# Autodesk Inventor assembly: rear_sled
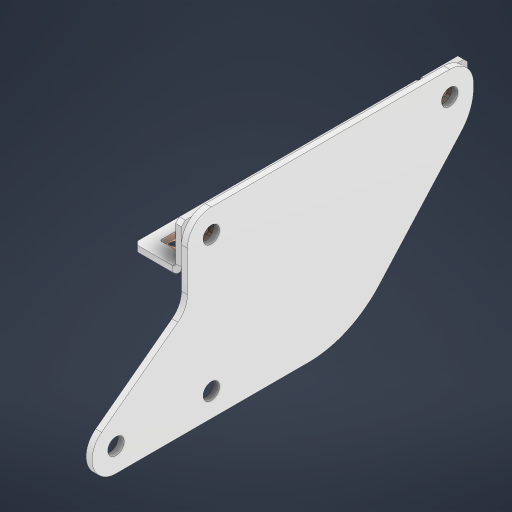
[picture p0: Inventor's stored thumbnail of the model, 512x512]
Saved by Autodesk Inventor 2024 (Build 280153000, 153)
## iProperties
Created: 2024-01-16
Part Number: rear_sled
Document SubType Name: Assembly
Designer: avere
Author: avere
## Documents named in this file (3)
- C:\Users\avere\Documents\rbp_cad\zoomba_v0.3\chassis\drivebay\rear_sled.iam
- C:\Users\avere\Documents\rbp_cad\zoomba_v0.3\chassis\drivebay\custom_parts\sled.ipt
- C:\Users\avere\Documents\rbp_cad\VEX-CAD-Inventor-1.41\Structure\Angle\Aluminum 1x1\Alu Angle 1x1x6.ipt
## Components (2 placed, 2 different names)
1. sled:1 — Insert:1, Mate:1
2. Alu Angle 1x1x6:1 — Insert:1, Mate:1
## Relationships (2: Insert 1, Mate 1)
- Insert:1: sled:1 ↔ Alu Angle 1x1x6:1
- Mate:1: sled:1 ↔ Alu Angle 1x1x6:1
